# Autodesk Inventor assembly: MultiPassSCAN_outsideIn-DFMOD_SCAN_COLOR_mechanical
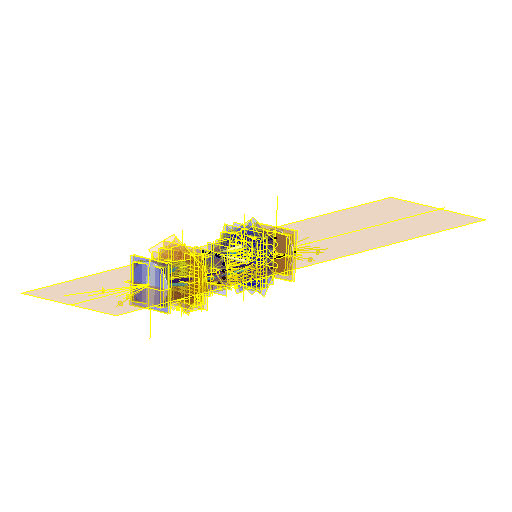
[picture p0: Inventor's stored thumbnail of the model, 512x512]
Saved by Autodesk Inventor 2026.1 (Build 301233000, 233)
## iProperties
Created: 2024-08-19
Part Number: MultiPassSCAN_outsideIn-DFMOD_SCAN_COLOR_mechanical
Document SubType Name: Assembly
Designer: User
Author: User
## Documents named in this file (16)
- C:\Users\farin012\Downloads\fig4\fig4\MultiPassSCAN_outsideIn-DFMOD_SCAN_COLOR_mechanical.iam
- C:\Users\farin012\Downloads\fig4\fig4\BB1-E02-Solidworks.ipt
- C:\Users\farin012\Downloads\fig4\fig4\LoopPlane1.ipt
- C:\Users\farin012\Downloads\fig4\fig4\LA1608-AB-Solidworks\LA1608-AB-2LOOP_grid.ipt
- C:\Users\farin012\Downloads\fig4\fig4\LOOP1_COLL.ipt
- C:\Users\farin012\Downloads\fig4\fig4\LOOP1_COLL_PREDEF1.ipt
- C:\Users\farin012\Downloads\fig4\fig4\deflection_plane.ipt
- C:\Users\farin012\Downloads\fig4\fig4\LOOP1_COLL_POSTDEF2.ipt
- C:\Users\farin012\Downloads\fig4\fig4\LOOP2_COLL_PREDEF1.ipt
- C:\Users\farin012\Downloads\fig4\fig4\LOOP2_COLL_POSTDEF2.ipt
- C:\Users\farin012\Downloads\fig4\fig4\LaserBeamEntry2_UNDEF.ipt
- C:\Users\farin012\Downloads\fig4\fig4\LaserBeamEntry2_LOOP1DEF2.ipt
- C:\Users\farin012\Downloads\fig4\fig4\LaserBeamEntry2_LOOP2DEF2.ipt
- C:\Users\farin012\Downloads\fig4\fig4\EntryMirror.ipt
- C:\Users\farin012\Downloads\fig4\fig4\ExitMirror.ipt
- C:\Users\farin012\Downloads\fig4\fig4\LaserBeamEntry2.ipt
## Components (28 placed, 15 different names)
1. BB1-E02-Solidworks:1 — Mate:115, Mate:125, Mate:126, Mate:127, Angle:6, Mate:128, Mate:147
2. BB1-E02-Solidworks:2 — Mate:233, Angle:9, Angle:10
3. LoopPlane1:1 — Mate:113
4. LA1608-AB-2LOOP_grid:1 — Flush:3, Mate:145, Mate:147, Mate:148, Mate:173, Mate:174, Mate:175, Mate:176, Mate:196, Flush:172, Mate:197, Flush:173, Mate:204, Flush:180, Mate:205, Flush:181
5. LA1608-AB-2LOOP_grid:2 — Flush:2, Mate:145, Mate:149, Mate:155, Mate:156, Mate:169, Mate:170, Mate:179, Mate:180, Mate:193, Mate:194, Mate:198, Flush:174, Mate:203, Flush:179, Mate:206, Flush:182, Mate:211, Flush:187
6. LOOP1_COLL:1 — Mate:125, Mate:126
7. LOOP1_COLL:2 — Mate:127, Mate:128
8. LOOP1_COLL_PREDEF1:1 — Mate:155, Mate:156
9. deflection_plane:1 — Mate:230, Flush:190, Angle:9
10. LOOP1_COLL_POSTDEF2:1 — Mate:169, Mate:170
11. LOOP2_COLL_PREDEF1:1 — Mate:173, Mate:174
12. LOOP2_COLL_PREDEF1:2 — Mate:175, Mate:176
13. LOOP2_COLL_PREDEF1:3 — Mate:179, Mate:180
14. LOOP2_COLL_POSTDEF2:1 — Mate:193, Mate:194
15. LaserBeamEntry2_UNDEF:1 — Mate:196, Flush:172, Mate:216, Mate:218, Mate:220, Mate:221
16. LaserBeamEntry2_UNDEF:2 — Mate:198, Flush:174
17. LaserBeamEntry2_UNDEF:3 — Mate:197, Flush:173
18. LaserBeamEntry2_LOOP1DEF2:1 — Mate:204, Flush:180
19. LaserBeamEntry2_LOOP1DEF2:2 — Mate:203, Flush:179
20. LaserBeamEntry2_LOOP1DEF2:3 — Mate:205, Flush:181
21. LaserBeamEntry2_LOOP1DEF2:4 — Mate:206, Flush:182
22. LaserBeamEntry2_LOOP2DEF2:1 — Mate:211, Flush:187, Mate:225
23. deflection_plane:2 — Mate:216, Mate:217, Mate:218, Mate:219, Mate:226
24. EntryMirror:1 — Mate:220, Angle:7, Mate:221, Mate:222, Flush:188
25. ExitMirror:1 — Mate:223, Mate:224, Mate:225, Flush:189
26. deflection_plane:3 — Mate:231, Angle:8
27. LaserBeamEntry2:1 — Mate:222, Flush:188
28. LaserBeamEntry2_LOOP2DEF2:2 — Mate:226, Flush:189
## Relationships (64: Mate 46, Flush 13, Angle 5)
- Mate:22
- Mate:23
- Mate:113: LoopPlane1:1
- Mate:115: BB1-E02-Solidworks:1
- Flush:2: LA1608-AB-2LOOP_grid:2
- Flush:3: LA1608-AB-2LOOP_grid:1
- Mate:125: BB1-E02-Solidworks:1 ↔ LOOP1_COLL:1
- Mate:126: BB1-E02-Solidworks:1 ↔ LOOP1_COLL:1
- Mate:127: BB1-E02-Solidworks:1 ↔ LOOP1_COLL:2
- Angle:6 (0 deg): BB1-E02-Solidworks:1
- Mate:128: BB1-E02-Solidworks:1 ↔ LOOP1_COLL:2
- Mate:145 (-50 mm): LA1608-AB-2LOOP_grid:1 ↔ LA1608-AB-2LOOP_grid:2
- Mate:147 (25 mm): BB1-E02-Solidworks:1 ↔ LA1608-AB-2LOOP_grid:1
- Mate:148: LA1608-AB-2LOOP_grid:1
- Mate:149: LA1608-AB-2LOOP_grid:2
- Mate:155: LA1608-AB-2LOOP_grid:2 ↔ LOOP1_COLL_PREDEF1:1
- Mate:156: LA1608-AB-2LOOP_grid:2 ↔ LOOP1_COLL_PREDEF1:1
- Mate:169: LA1608-AB-2LOOP_grid:2 ↔ LOOP1_COLL_POSTDEF2:1
- Mate:170: LA1608-AB-2LOOP_grid:2 ↔ LOOP1_COLL_POSTDEF2:1
- Mate:173: LA1608-AB-2LOOP_grid:1 ↔ LOOP2_COLL_PREDEF1:1
- Mate:174: LA1608-AB-2LOOP_grid:1 ↔ LOOP2_COLL_PREDEF1:1
- Mate:175: LA1608-AB-2LOOP_grid:1 ↔ LOOP2_COLL_PREDEF1:2
- Mate:176: LA1608-AB-2LOOP_grid:1 ↔ LOOP2_COLL_PREDEF1:2
- Mate:179: LA1608-AB-2LOOP_grid:2 ↔ LOOP2_COLL_PREDEF1:3
- Mate:180: LA1608-AB-2LOOP_grid:2 ↔ LOOP2_COLL_PREDEF1:3
- Mate:193: LA1608-AB-2LOOP_grid:2 ↔ LOOP2_COLL_POSTDEF2:1
- Mate:194: LA1608-AB-2LOOP_grid:2 ↔ LOOP2_COLL_POSTDEF2:1
- Mate:196: LA1608-AB-2LOOP_grid:1 ↔ LaserBeamEntry2_UNDEF:1
- Flush:172: LA1608-AB-2LOOP_grid:1 ↔ LaserBeamEntry2_UNDEF:1
- Mate:197: LA1608-AB-2LOOP_grid:1 ↔ LaserBeamEntry2_UNDEF:3
- Mate:198: LA1608-AB-2LOOP_grid:2 ↔ LaserBeamEntry2_UNDEF:2
- Flush:173: LA1608-AB-2LOOP_grid:1 ↔ LaserBeamEntry2_UNDEF:3
- Flush:174: LA1608-AB-2LOOP_grid:2 ↔ LaserBeamEntry2_UNDEF:2
- Mate:203: LA1608-AB-2LOOP_grid:2 ↔ LaserBeamEntry2_LOOP1DEF2:2
- Flush:179: LA1608-AB-2LOOP_grid:2 ↔ LaserBeamEntry2_LOOP1DEF2:2
- Mate:204: LA1608-AB-2LOOP_grid:1 ↔ LaserBeamEntry2_LOOP1DEF2:1
- Flush:180: LA1608-AB-2LOOP_grid:1 ↔ LaserBeamEntry2_LOOP1DEF2:1
- Mate:205: LA1608-AB-2LOOP_grid:1 ↔ LaserBeamEntry2_LOOP1DEF2:3
- Flush:181: LA1608-AB-2LOOP_grid:1 ↔ LaserBeamEntry2_LOOP1DEF2:3
- Mate:206: LA1608-AB-2LOOP_grid:2 ↔ LaserBeamEntry2_LOOP1DEF2:4
- Flush:182: LA1608-AB-2LOOP_grid:2 ↔ LaserBeamEntry2_LOOP1DEF2:4
- Mate:211: LA1608-AB-2LOOP_grid:2 ↔ LaserBeamEntry2_LOOP2DEF2:1
- Flush:187: LA1608-AB-2LOOP_grid:2 ↔ LaserBeamEntry2_LOOP2DEF2:1
- Mate:216: LaserBeamEntry2_UNDEF:1 ↔ deflection_plane:2
- Mate:217: deflection_plane:2
- Mate:218: LaserBeamEntry2_UNDEF:1 ↔ deflection_plane:2
- Mate:219: deflection_plane:2
- Mate:220: LaserBeamEntry2_UNDEF:1 ↔ EntryMirror:1
- Angle:7 (180 deg): EntryMirror:1
- Mate:221: LaserBeamEntry2_UNDEF:1 ↔ EntryMirror:1
- Mate:222: EntryMirror:1 ↔ LaserBeamEntry2:1
- Flush:188: EntryMirror:1 ↔ LaserBeamEntry2:1
- Mate:223: ExitMirror:1
- Mate:224: ExitMirror:1
- Mate:225: LaserBeamEntry2_LOOP2DEF2:1 ↔ ExitMirror:1
- Mate:226: deflection_plane:2 ↔ LaserBeamEntry2_LOOP2DEF2:2
- Flush:189: ExitMirror:1 ↔ LaserBeamEntry2_LOOP2DEF2:2
- Mate:230: deflection_plane:1
- Flush:190: deflection_plane:1
- Mate:231: deflection_plane:3
- Angle:8 (90 deg): deflection_plane:3
- Mate:233: BB1-E02-Solidworks:2
- Angle:9 (90 deg): BB1-E02-Solidworks:2 ↔ deflection_plane:1
- Angle:10 (175 deg): BB1-E02-Solidworks:2
